# Autodesk Inventor assembly: RCUv2-2Assy
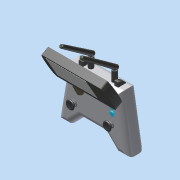
[picture p0: Inventor's stored thumbnail of the model, 180x180]
Saved by Autodesk Inventor 2011 SP1 (Build 150282100, 282)
## iProperties
Created: 2011-08-14
Part Number: RCUv2-2Assy
Document SubType Name: Assembly
Designer: dgitz
Author: dgitz
## Documents named in this file (4)
- C:\Dropbox\ICARUS\Remote Control Unit (RCU)\RCU v2\Design\RCUv2-2Assy.iam
- C:\Dropbox\ICARUS\Remote Control Unit (RCU)\RCU v2\Design\Library\SpringSamsungGalaxySAssy.iam
- C:\Dropbox\ICARUS\Remote Control Unit (RCU)\RCU v2\Design\Library\XBeeAntennaAssy.iam
- C:\Dropbox\ICARUS\Remote Control Unit (RCU)\RCU v2\Design\RCUv2-2\RCUAssy.iam
## Components (4 placed, 3 different names)
1. SpringSamsungGalaxySAssy:1 [sub-assembly] — Mate:1, Angle:1
2. XBeeAntennaAssy:1 [sub-assembly] — Mate:2, Mate:4, Mate:5
3. XBeeAntennaAssy:2 [sub-assembly] — Mate:3, Mate:4, Mate:5
4. RCUAssy:1 [sub-assembly] — Mate:1, Angle:1, Mate:2, Mate:3
## Relationships (6: Mate 5, Angle 1)
- Mate:1: SpringSamsungGalaxySAssy:1 ↔ RCUAssy:1
- Angle:1 (150 deg): SpringSamsungGalaxySAssy:1 ↔ RCUAssy:1
- Mate:2: XBeeAntennaAssy:1 ↔ RCUAssy:1
- Mate:3: XBeeAntennaAssy:2 ↔ RCUAssy:1
- Mate:4 (50.8 mm): XBeeAntennaAssy:1 ↔ XBeeAntennaAssy:2
- Mate:5 (50.8 mm): XBeeAntennaAssy:1 ↔ XBeeAntennaAssy:2
